# Autodesk Inventor assembly: Piece_L
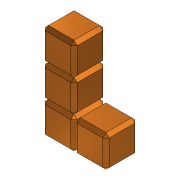
[picture p0: Inventor's stored thumbnail of the model, 180x180]
Saved by Autodesk Inventor 2021 (Build 250183000, 183)
## iProperties
Created: 2021-04-01
Part Number: Piece_L
Document SubType Name: Assembly
Designer: Tran Duc Viet
Mass: 9122.47 g
Surface Area: 526.693 cm^2
Volume: 472.667 cm^3
Density: 19.3 g/cm^3
Author: Tran Duc Viet
## Documents named in this file (2)
- C:\Users\davei\Desktop\School\Léto 2020-2021\VRM\Projects\P2\Piece_L.iam
- C:\Users\davei\Desktop\School\Léto 2020-2021\VRM\Projects\P2\ElementaryCube_GOLD.ipt
## Components (4 placed, 1 different names)
1. ElementaryCube_GOLD:1 — Mate:1, Flush:1, Flush:2, Mate:2, Flush:3, Flush:4
2. ElementaryCube_GOLD:2 — Mate:3, Flush:5, Flush:6
3. ElementaryCube_GOLD:3 — Mate:2, Flush:3, Flush:4, Mate:3, Flush:5, Flush:6
4. ElementaryCube_GOLD:4 — Mate:1, Flush:1, Flush:2
## Relationships (9: Flush 6, Mate 3)
- Mate:1: ElementaryCube_GOLD:1 ↔ ElementaryCube_GOLD:4
- Flush:1: ElementaryCube_GOLD:1 ↔ ElementaryCube_GOLD:4
- Flush:2: ElementaryCube_GOLD:1 ↔ ElementaryCube_GOLD:4
- Mate:2: ElementaryCube_GOLD:1 ↔ ElementaryCube_GOLD:3
- Flush:3: ElementaryCube_GOLD:1 ↔ ElementaryCube_GOLD:3
- Flush:4: ElementaryCube_GOLD:1 ↔ ElementaryCube_GOLD:3
- Mate:3: ElementaryCube_GOLD:2 ↔ ElementaryCube_GOLD:3
- Flush:5: ElementaryCube_GOLD:2 ↔ ElementaryCube_GOLD:3
- Flush:6: ElementaryCube_GOLD:2 ↔ ElementaryCube_GOLD:3
